(part 1 of 2)
# Autodesk Inventor assembly: gasienica_zlozenie
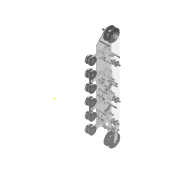
[picture p0: Inventor's stored thumbnail of the model, 180x180]
Saved by Autodesk Inventor 2020.3 (Build 243373000, 373)
## iProperties
Created: 2021-10-24
Part Number: gasienica_zlozenie
Document SubType Name: Assembly
Designer: Patryk Szydlik
Project: Projekt gąsienicowego układu jezdnego robota mobilnego "Ariadna"
Description: Projekt gąsienicowego układu jezdnego robota mobilnego "Ariadna"
Author: Patryk Szydlik
Title: Projekt gąsienicowego układu jezdnego robota mobilnego "Ariadna"
Subject: Projekt gąsienicowego układu jezdnego robota mobilnego "Ariadna"
## Documents named in this file (48)
- C:\Users\patry\Desktop\Semestr 7\Inzynierka\Projekt inventor\Ariadna_inzynierka\Workspaces\Obszar roboczy\Obszar roboczy\Naped\Zawieszenie_v3\gasienica_zlozenie.iam
- C:\Users\patry\Desktop\Semestr 7\Inzynierka\Projekt inventor\Ariadna_inzynierka\Workspaces\Obszar roboczy\Obszar roboczy\Naped\Kola\kolo_przednie.iam
- C:\Users\patry\Desktop\Semestr 7\Inzynierka\Projekt inventor\Ariadna_inzynierka\Workspaces\Obszar roboczy\Obszar roboczy\Naped\Sruby\M5x65.ipt
- C:\Users\patry\Desktop\Semestr 7\Inzynierka\Projekt inventor\Ariadna_inzynierka\Workspaces\Obszar roboczy\Obszar roboczy\Naped\Sruby\M5_nut_5mm.ipt
- C:\Users\patry\Desktop\Semestr 7\Inzynierka\Projekt inventor\Ariadna_inzynierka\Workspaces\Obszar roboczy\Obszar roboczy\Naped\Sruby\dystans_miedzy_plytami.ipt
- C:\Users\patry\Desktop\Semestr 7\Inzynierka\Projekt inventor\Ariadna_inzynierka\Workspaces\Obszar roboczy\Obszar roboczy\Naped\Zawieszenie_v3\tuleja_TUF106040.ipt
- C:\Users\patry\Desktop\Semestr 7\Inzynierka\Projekt inventor\Ariadna_inzynierka\Workspaces\Obszar roboczy\Obszar roboczy\Naped\Sruby\M6_nut_5mm.ipt
- C:\Users\patry\Desktop\Semestr 7\Inzynierka\Projekt inventor\Ariadna_inzynierka\Workspaces\Obszar roboczy\Obszar roboczy\Naped\Amortyzator\Korpus.ipt
- C:\Users\patry\Desktop\Semestr 7\Inzynierka\Projekt inventor\Ariadna_inzynierka\Workspaces\Obszar roboczy\Obszar roboczy\Naped\Amortyzator\Tlok.ipt
- C:\Users\patry\Desktop\Semestr 7\Inzynierka\Projekt inventor\Ariadna_inzynierka\Workspaces\Obszar roboczy\Obszar roboczy\Naped\Amortyzator\Nakretka.ipt
- C:\Users\patry\Desktop\Semestr 7\Inzynierka\Projekt inventor\Ariadna_inzynierka\Workspaces\Obszar roboczy\Obszar roboczy\Naped\Sruby\M8_nut_6.5mm_MIR1.ipt
- C:\Users\patry\Desktop\Semestr 7\Inzynierka\Projekt inventor\Ariadna_inzynierka\Workspaces\Obszar roboczy\Obszar roboczy\Naped\Sruby\M8x80_threaded_MIR1.ipt
- C:\Users\patry\Desktop\Semestr 7\Inzynierka\Projekt inventor\Ariadna_inzynierka\Workspaces\Obszar roboczy\Obszar roboczy\Naped\Sruby\M8_pad_MIR1.ipt
- C:\Users\patry\Desktop\Semestr 7\Inzynierka\Projekt inventor\Ariadna_inzynierka\Workspaces\Obszar roboczy\Obszar roboczy\Naped\Lozyska\608ZZ-8mm\bearings-608zz-80018-1.snapshot.1\608zz_MIR1.ipt
- C:\Users\patry\Desktop\Semestr 7\Inzynierka\Projekt inventor\Ariadna_inzynierka\Workspaces\Obszar roboczy\Obszar roboczy\Naped\Kola\kolo_napedowe.iam
- C:\Users\patry\Desktop\Semestr 7\Inzynierka\Projekt inventor\Ariadna_inzynierka\Workspaces\Obszar roboczy\Obszar roboczy\Naped\Sruby\M5_70_shaft.ipt
- C:\Users\patry\Desktop\Semestr 7\Inzynierka\Projekt inventor\Ariadna_inzynierka\Workspaces\Obszar roboczy\Obszar roboczy\Naped\Sruby\M3_16_shaft.ipt
- C:\Users\patry\Desktop\Semestr 7\Inzynierka\Projekt inventor\Ariadna_inzynierka\Workspaces\Obszar roboczy\Obszar roboczy\Naped\Sruby\M3_nut_2,5mm.ipt
- C:\Users\patry\Desktop\Semestr 7\Inzynierka\Projekt inventor\Ariadna_inzynierka\Workspaces\Obszar roboczy\Obszar roboczy\Naped\Zawieszenie_v3\wspornik_amortyzatora.ipt
- C:\Users\patry\Desktop\Semestr 7\Inzynierka\Projekt inventor\Ariadna_inzynierka\Workspaces\Obszar roboczy\Obszar roboczy\Naped\Sruby\M6_70_shaft.ipt
- C:\Users\patry\Desktop\Semestr 7\Inzynierka\Projekt inventor\Ariadna_inzynierka\Workspaces\Obszar roboczy\Obszar roboczy\Naped\Sruby\tuleja_M5_M9_20.ipt
- C:\Users\patry\Desktop\Semestr 7\Inzynierka\Projekt inventor\Ariadna_inzynierka\Workspaces\Obszar roboczy\Obszar roboczy\Naped\Sruby\tuleja_M5_M9_25.ipt
- C:\Users\patry\Desktop\Semestr 7\Inzynierka\Projekt inventor\Ariadna_inzynierka\Workspaces\Obszar roboczy\Obszar roboczy\Naped\Kola\holder_wheel_pair.iam
- C:\Users\patry\Desktop\Semestr 7\Inzynierka\Projekt inventor\Ariadna_inzynierka\Workspaces\Obszar roboczy\Obszar roboczy\Naped\Zawieszenie_v3\ramie_napinacza.ipt
- C:\Users\patry\Desktop\Semestr 7\Inzynierka\Projekt inventor\Ariadna_inzynierka\Workspaces\Obszar roboczy\Obszar roboczy\Naped\Sruby\M5_60_shaft.ipt
- C:\Users\patry\Desktop\Semestr 7\Inzynierka\Projekt inventor\Ariadna_inzynierka\Workspaces\Obszar roboczy\Obszar roboczy\Naped\Sruby\tuleja_M5_M9_13.ipt
- C:\Users\patry\Desktop\Semestr 7\Inzynierka\Projekt inventor\Ariadna_inzynierka\Workspaces\Obszar roboczy\Obszar roboczy\Naped\Sruby\tuleja_M5_M9_18.ipt
- C:\Users\patry\Desktop\Semestr 7\Inzynierka\Projekt inventor\Ariadna_inzynierka\Workspaces\Obszar roboczy\Obszar roboczy\Naped\Sruby\tuleja_M6_M10_8.ipt
- C:\Users\patry\Desktop\Semestr 7\Inzynierka\Projekt inventor\Ariadna_inzynierka\Workspaces\Obszar roboczy\Obszar roboczy\Naped\Zawieszenie_v3\plyta_boczna.ipt
- C:\Users\patry\Desktop\Semestr 7\Inzynierka\Projekt inventor\Ariadna_inzynierka\Workspaces\Obszar roboczy\Obszar roboczy\Naped\Zawieszenie_v3\ramie_1_wahacza.ipt
- C:\Users\patry\Desktop\Semestr 7\Inzynierka\Projekt inventor\Ariadna_inzynierka\Workspaces\Obszar roboczy\Obszar roboczy\Naped\Zawieszenie_v3\ramie_2_wahacza.ipt
- C:\Users\patry\Desktop\Semestr 7\Inzynierka\Projekt inventor\Ariadna_inzynierka\Workspaces\Obszar roboczy\Obszar roboczy\Naped\Sruby\M6_40_shaft.ipt
- C:\Users\patry\Desktop\Semestr 7\Inzynierka\Projekt inventor\Ariadna_inzynierka\Workspaces\Obszar roboczy\Obszar roboczy\Naped\Sruby\tuleja_M6_M10_7.ipt
- C:\Users\patry\Desktop\Semestr 7\Inzynierka\Projekt inventor\Ariadna_inzynierka\Workspaces\Obszar roboczy\Obszar roboczy\Naped\Sruby\M6_1,25_pad.ipt
- C:\Users\patry\Desktop\Semestr 7\Inzynierka\Projekt inventor\Ariadna_inzynierka\Workspaces\Obszar roboczy\Obszar roboczy\Naped\Sruby\M5_40_shaft.ipt
- M5_shaft.ipt
- C:\Users\patry\Desktop\Semestr 7\Inzynierka\Projekt inventor\Ariadna_inzynierka\Workspaces\Obszar roboczy\Obszar roboczy\Naped\Sruby\tuleja_M5_M9_4,5.ipt
- C:\Users\patry\Desktop\Semestr 7\Inzynierka\Projekt inventor\Ariadna_inzynierka\Workspaces\Obszar roboczy\Obszar roboczy\Naped\Zawieszenie_v3\glowny_wahacz_zewn.ipt
- C:\Users\patry\Desktop\Semestr 7\Inzynierka\Projekt inventor\Ariadna_inzynierka\Workspaces\Obszar roboczy\Obszar roboczy\Naped\Zawieszenie_v3\independent_wheel_pair.iam
- C:\Users\patry\Desktop\Semestr 7\Inzynierka\Projekt inventor\Ariadna_inzynierka\Workspaces\Obszar roboczy\Obszar roboczy\Naped\Sruby\tuleja_M6_M10_6.ipt
- C:\Users\patry\Desktop\Semestr 7\Inzynierka\Projekt inventor\Ariadna_inzynierka\Workspaces\Obszar roboczy\Obszar roboczy\Naped\Sruby\tuleja_M5_M9_17.5.ipt
- C:\Users\patry\Desktop\Semestr 7\Inzynierka\Projekt inventor\Ariadna_inzynierka\Workspaces\Obszar roboczy\Obszar roboczy\Naped\Zawieszenie_v3\komplet_kol_V4.iam
- C:\Users\patry\Desktop\Semestr 7\Inzynierka\Projekt inventor\Ariadna_inzynierka\Workspaces\Obszar roboczy\Obszar roboczy\Naped\Sruby\M6_25_shaft.ipt
- C:\Users\patry\Desktop\Semestr 7\Inzynierka\Projekt inventor\Ariadna_inzynierka\Workspaces\Obszar roboczy\Obszar roboczy\Naped\Kola\single_wheel_dummie.iam
- C:\Users\patry\Desktop\Semestr 7\Inzynierka\Projekt inventor\Ariadna_inzynierka\Workspaces\Obszar roboczy\Obszar roboczy\Naped\Sruby\tuleja_M5_M10_15.ipt
- C:\Users\patry\Desktop\Semestr 7\Inzynierka\Projekt inventor\Ariadna_inzynierka\Workspaces\Obszar roboczy\Obszar roboczy\Naped\Sruby\tuleja_M6_M10_7,5.ipt
- C:\Users\patry\Desktop\Semestr 7\Inzynierka\Projekt inventor\Ariadna_inzynierka\Workspaces\Obszar roboczy\Obszar roboczy\Naped\Zawieszenie_v3\ramie_2_wahacza_tylnego.ipt
- C:\Users\patry\Desktop\Semestr 7\Inzynierka\Projekt inventor\Ariadna_inzynierka\Workspaces\Obszar roboczy\Obszar roboczy\Naped\Sruby\M6x25_plaski_leb.ipt
## Components (346 placed, 46 different names)
1. M5x65:3 — Zestawiające:1808, Zestawiające:1809, Zestawiające:1810
2. M5_nut_5mm:3 — Zestawiające:1810, Zestawiające:1811
3. dystans_miedzy_plytami:3
4. M8_nut_6.5mm_MIR1:1
5. M8x80_threaded_MIR1:1
6. M8_nut_6.5mm_MIR1:2
7. M8_nut_6.5mm_MIR1:3
8. M8_pad_MIR1:1
9. M8_pad_MIR1:2
10. M8_pad_MIR1:3
11. M8_pad_MIR1:4
12. 608zz_MIR1:1
13. 608zz_MIR1:2 — Zestawiające:1077, Równoległe:74
14. kolo_napedowe:1 [sub-assembly]
15. kolo_przednie:1 [sub-assembly]
16. ramie_napinacza:1 — Zestawiające:1807
17. Korpus:6 — Walcowe:6
18. Tlok:6 — Walcowe:6
19. Nakretka:6
20. M5_nut_5mm:34
21. M5_70_shaft:6 — Zestawiające:1080
22. M5_nut_5mm:35
23. M3_16_shaft:6
24. M3_nut_2,5mm:11
25. M3_nut_2,5mm:12
26. wspornik_amortyzatora:11 — Zestawiające:1086, Zestawiające:1087
27. wspornik_amortyzatora:12
28. M5_nut_5mm:36
29. M5_nut_5mm:37
30. M5_nut_5mm:38
31. M5_nut_5mm:39
32. tuleja_M5_M9_20:6
33. tuleja_M5_M9_25:6
34. ramie_napinacza:2 — Zestawiające:1804
35. M5_60_shaft:1 — Zestawiające:1086
36. M5_60_shaft:2 — Zestawiające:1087, Zestawiające:1796, Zestawiające:1797
37. tuleja_TUF106040:41 — Zestawiające:1085
38. tuleja_TUF106040:42
39. M6_70_shaft:11 — Zestawiające:1079, Zestawiające:1802, Zestawiające:1803, Zestawiające:1806
40. M6_nut_5mm:49
41. M6_nut_5mm:50
42. tuleja_M5_M9_13:1 — Zestawiające:1796
43. tuleja_M5_M9_18:1 — Zestawiające:1797
44. M6_70_shaft:12
45. M6_nut_5mm:51
46. M6_nut_5mm:52
47. tuleja_M6_M10_8:1
48. tuleja_M6_M10_8:2
49. holder_wheel_pair:4 [sub-assembly] — Zestawiające:1082, Zestawiające:1083
50. holder_wheel_pair:5 [sub-assembly] — Zestawiające:1081, Zestawiające:1084
51. plyta_boczna:1 — Zestawiające:1075, Zestawiające:1076, Zestawiające:1077, Zestawiające:1078, Równoległe:74, Kątowe:22, Zestawiające:1079, Zestawiające:1080, Zestawiające:1081, Zestawiające:1082, Zestawiające:1083, Zestawiające:1084, Zestawiające:1085, Zestawiające:1632, Zestawiające:1633, Kątowe:49, Zestawiające:1808, Zestawiające:1809, Zestawiające:1950, Zestawiające:1951, Zestawiające:1952, Zestawiające:1953
52. plyta_boczna:2 — Zestawiające:1075, Zestawiające:1076, Zestawiające:1078, Zestawiające:1636, Zestawiające:1637, Zestawiające:1638, Zestawiające:1639, Zestawiające:1640, Zestawiające:1641, Zestawiające:1777, Zestawiające:1778, Zestawiające:1779, Zestawiające:1780, Zestawiające:1811
53. ramie_1_wahacza:3
54. ramie_2_wahacza:3
55. tuleja_TUF106040:51
56. tuleja_TUF106040:52
57. tuleja_TUF106040:53
58. tuleja_TUF106040:54
59. tuleja_TUF106040:55
60. tuleja_TUF106040:56
61. ramie_2_wahacza:4
62. tuleja_TUF106040:57
63. tuleja_TUF106040:58
64. M6_nut_5mm:65
65. Korpus:8
66. Tlok:8
67. Nakretka:8
68. M5_nut_5mm:48
69. M5_70_shaft:8
70. ramie_1_wahacza:4 — Kątowe:40
71. M5_nut_5mm:49
72. M3_16_shaft:8
73. M3_nut_2,5mm:15
74. M3_nut_2,5mm:16
75. wspornik_amortyzatora:15
76. wspornik_amortyzatora:16
77. M6_40_shaft:3
78. M6_40_shaft:4
79. M6_nut_5mm:66
80. M6_nut_5mm:67
81. M6_nut_5mm:68
82. tuleja_M6_M10_7:4
83. tuleja_M6_M10_7:5
84. M6_1,25_pad:9
85. M6_1,25_pad:10
86. M6_1,25_pad:11
87. M6_1,25_pad:12
88. M6_1,25_pad:13
89. M6_1,25_pad:14
90. M6_1,25_pad:15
91. M6_1,25_pad:16
92. M6_70_shaft:15 — Zestawiające:1636
93. M6_70_shaft:16 — Zestawiające:1632
94. M6_nut_5mm:69
95. M6_nut_5mm:70
96. M6_nut_5mm:71
97. M6_nut_5mm:72
98. M5_shaft:3
99. M5_shaft:4
100. M5_nut_5mm:50
101. M5_nut_5mm:51
102. M5_nut_5mm:52
103. M5_nut_5mm:53
104. tuleja_M5_M9_4,5:5
105. tuleja_M5_M9_4,5:6
106. tuleja_M5_M9_4,5:7
107. tuleja_M5_M9_4,5:8
108. lacznik_zewn:3 — Kątowe:40, Zestawiające:1793, Zestawiające:1794, Zestawiające:1795
109. lacznik_zewn:4 — Zestawiające:1793
110. tuleja_M6_M10_6:5
111. M6_nut_5mm:73
112. M6_nut_5mm:74
113. M6_nut_5mm:75 — Zestawiające:1633
114. M6_nut_5mm:76
115. tuleja_M6_M10_6:6
116. tuleja_M6_M10_6:7
117. tuleja_M6_M10_6:8
118. M5_nut_5mm:54
119. M5_nut_5mm:55
120. tuleja_M5_M9_17.5:3 — Zestawiające:1637
121. tuleja_M5_M9_17.5:4
122. ramie_1_wahacza:7 — Kątowe:41
123. ramie_2_wahacza:7
124. tuleja_TUF106040:67
125. tuleja_TUF106040:68
126. tuleja_TUF106040:69
127. tuleja_TUF106040:70
128. tuleja_TUF106040:71
129. tuleja_TUF106040:72
130. ramie_2_wahacza:8
131. tuleja_TUF106040:73
132. tuleja_TUF106040:74
133. M6_nut_5mm:89
134. Korpus:10 — Walcowe:10
135. Tlok:10 — Walcowe:10
136. Nakretka:10
137. M5_nut_5mm:64
138. M5_70_shaft:10
139. ramie_1_wahacza:8
140. M5_nut_5mm:65 — Zestawiające:1638
141. M3_16_shaft:10
142. M3_nut_2,5mm:19
143. M3_nut_2,5mm:20
144. wspornik_amortyzatora:19
145. wspornik_amortyzatora:20
146. M6_40_shaft:7
147. M6_40_shaft:8
148. M6_nut_5mm:90
149. M6_nut_5mm:91
150. M6_nut_5mm:92
151. tuleja_M6_M10_7:10
152. tuleja_M6_M10_7:11
153. M6_1,25_pad:25
154. M6_1,25_pad:26
155. M6_1,25_pad:27
156. M6_1,25_pad:28
157. M6_1,25_pad:29
158. M6_1,25_pad:30
159. M6_1,25_pad:31
160. M6_1,25_pad:32
161. M6_70_shaft:19 — Zestawiające:1640
162. M6_70_shaft:20 — Zestawiające:1639
163. M6_nut_5mm:93
164. M6_nut_5mm:94
165. M6_nut_5mm:95
166. M6_nut_5mm:96
167. M5_shaft:7
168. M5_shaft:8
169. M5_nut_5mm:66
170. M5_nut_5mm:67
171. M5_nut_5mm:68
172. M5_nut_5mm:69
173. tuleja_M5_M9_4,5:13
174. tuleja_M5_M9_4,5:14
175. tuleja_M5_M9_4,5:15
176. tuleja_M5_M9_4,5:16
177. lacznik_zewn:7 — Zestawiające:1784
178. lacznik_zewn:8 — Kątowe:41, Zestawiające:1781, Zestawiające:1782, Zestawiające:1789
179. tuleja_M6_M10_6:13
180. M6_nut_5mm:97
181. M6_nut_5mm:98
182. M6_nut_5mm:99
183. M6_nut_5mm:100
184. tuleja_M6_M10_6:14
185. tuleja_M6_M10_6:15
186. tuleja_M6_M10_6:16
187. M5_nut_5mm:70
188. M5_nut_5mm:71
189. tuleja_M5_M9_17.5:7 — Zestawiające:1641
190. tuleja_M5_M9_17.5:8
191. ramie_1_wahacza:9 — Kątowe:47
192. ramie_2_wahacza:9
193. tuleja_TUF106040:75
194. tuleja_TUF106040:76
195. tuleja_TUF106040:77
196. tuleja_TUF106040:78
197. tuleja_TUF106040:79
198. tuleja_TUF106040:80
199. ramie_2_wahacza:10
200. tuleja_TUF106040:81
201. tuleja_TUF106040:82
202. M6_nut_5mm:101
203. Korpus:11 — Walcowe:11
204. Tlok:11 — Walcowe:11
205. Nakretka:11
206. M5_nut_5mm:72
207. M5_70_shaft:11
208. ramie_1_wahacza:10
209. M5_nut_5mm:73
210. M3_16_shaft:11
211. M3_nut_2,5mm:21
212. M3_nut_2,5mm:22
213. wspornik_amortyzatora:21
214. wspornik_amortyzatora:22
215. M6_40_shaft:9
216. M6_40_shaft:10
217. M6_nut_5mm:102
218. M6_nut_5mm:103
219. M6_nut_5mm:104
220. tuleja_M6_M10_7:13
221. tuleja_M6_M10_7:14
222. M6_1,25_pad:33
223. M6_1,25_pad:34
224. M6_1,25_pad:35
225. M6_1,25_pad:36
226. M6_1,25_pad:37
227. M6_1,25_pad:38
228. M6_1,25_pad:39
229. M6_1,25_pad:40
230. M6_70_shaft:21 — Zestawiające:1779
231. M6_70_shaft:22 — Zestawiające:1778
232. M6_nut_5mm:105
233. M6_nut_5mm:106
234. M6_nut_5mm:107 — Zestawiające:1777
235. M6_nut_5mm:108
236. M5_shaft:9
237. M5_shaft:10
238. M5_nut_5mm:74
239. M5_nut_5mm:75
240. M5_nut_5mm:76
241. M5_nut_5mm:77
242. tuleja_M5_M9_4,5:17
243. tuleja_M5_M9_4,5:18
244. tuleja_M5_M9_4,5:19
245. tuleja_M5_M9_4,5:20
246. lacznik_zewn:9
247. lacznik_zewn:10 — Kątowe:47
248. independent_wheel_pair:5 [sub-assembly]
249. tuleja_M6_M10_7:15
250. tuleja_M6_M10_6:17
251. M6_nut_5mm:109
252. M6_nut_5mm:110
253. M6_nut_5mm:111
254. M6_nut_5mm:112
255. tuleja_M6_M10_6:18
256. tuleja_M6_M10_6:19
257. tuleja_M6_M10_6:20
258. M5_nut_5mm:78
259. M5_nut_5mm:79
260. tuleja_M5_M9_17.5:9
261. tuleja_M5_M9_17.5:10 — Zestawiające:1780
262. komplet_kol_V4:1 [sub-assembly] — Zestawiające:1781, Zestawiające:1782, Zestawiające:1784, Zestawiające:1788, Kątowe:48
263. M6_nut_5mm:115 — Zestawiające:1789
264. M6_25_shaft:2 — Zestawiające:1788
265. M6_nut_5mm:116
266. komplet_kol_V4:2 [sub-assembly] — Zestawiające:1795, Kątowe:48, Kątowe:49, Styczny:1
267. M6_nut_5mm:117
268. M6_25_shaft:3 — Zestawiające:1794
269. M6_nut_5mm:118
270. single_wheel_dummie:1 [sub-assembly] — Zestawiające:1799
271. single_wheel_dummie:2 [sub-assembly] — Zestawiające:1800, Zestawiające:1801, Zestawiające:1802, Zestawiające:1805
272. tuleja_M5_M10_15:1 — Zestawiające:1799, Zestawiające:1800, Zestawiające:1801
273. tuleja_M6_M10_7,5:1 — Zestawiające:1803, Zestawiające:1804, Zestawiające:1805
274. tuleja_M6_M10_7,5:2 — Zestawiające:1806, Zestawiające:1807
275. ramie_1_wahacza:11
276. tuleja_TUF106040:83
277. tuleja_TUF106040:84
278. tuleja_TUF106040:85
279. tuleja_TUF106040:86
280. tuleja_TUF106040:87
281. tuleja_TUF106040:88
282. tuleja_TUF106040:89
283. tuleja_TUF106040:90
284. M6_nut_5mm:119
285. Korpus:12 — Walcowe:12
286. Tlok:12 — Walcowe:12
287. Nakretka:12
288. M5_nut_5mm:80
289. M5_70_shaft:12
290. ramie_1_wahacza:12
291. M5_nut_5mm:81
292. M3_16_shaft:12
293. M3_nut_2,5mm:23
294. M3_nut_2,5mm:24
295. wspornik_amortyzatora:23
296. wspornik_amortyzatora:24
297. M6_40_shaft:11
298. M6_40_shaft:12
299. M6_nut_5mm:120
300. M6_nut_5mm:121
301. M6_nut_5mm:122
302. tuleja_M6_M10_7:16
303. tuleja_M6_M10_7:17
304. M6_1,25_pad:41
305. M6_1,25_pad:42
306. M6_1,25_pad:43
307. M6_1,25_pad:44
308. M6_1,25_pad:45
309. M6_1,25_pad:46
310. M6_1,25_pad:47
311. M6_1,25_pad:48
312. M6_70_shaft:23 — Zestawiające:1950
313. M6_nut_5mm:123 — Zestawiające:1951
314. M6_nut_5mm:124
315. M6_nut_5mm:125
316. M6_nut_5mm:126
317. M5_shaft:11
318. M5_shaft:12
319. M5_nut_5mm:82
320. M5_nut_5mm:83
321. M5_nut_5mm:84
322. M5_nut_5mm:85
323. tuleja_M5_M9_4,5:21
324. tuleja_M5_M9_4,5:22
325. tuleja_M5_M9_4,5:23
326. tuleja_M5_M9_4,5:24
327. lacznik_zewn:11
328. lacznik_zewn:12
329. independent_wheel_pair:6 [sub-assembly] — Styczny:1
330. tuleja_M6_M10_7:18
331. tuleja_M6_M10_6:21
332. M6_nut_5mm:127
333. M6_nut_5mm:128
334. M6_nut_5mm:129
335. M6_nut_5mm:130
336. tuleja_M6_M10_6:22 — Zestawiające:1952
337. tuleja_M6_M10_6:23
338. tuleja_M6_M10_6:24
339. M5_nut_5mm:86
340. M5_nut_5mm:87
341. tuleja_M5_M9_17.5:11
342. tuleja_M5_M9_17.5:12 — Zestawiające:1953
343. ramie_2_wahacza_tylnego:1
344. ramie_2_wahacza_tylnego:2
345. M6x25_plaski_leb:1
346. M6x25_plaski_leb:2
## Relationships (744: Mate 670, Flush 48, Angle 21, CylindricalJoint 4, Tangent 1)
- [Mate]: M5x65:3 ↔ dystans_miedzy_plytami:3
- [Mate] (5 mm): M5x65:3 ↔ dystans_miedzy_plytami:3
- [Mate]: M8_nut_6.5mm_MIR1:1 ↔ M8x80_threaded_MIR1:1
- [Mate]: M8x80_threaded_MIR1:1 ↔ M8_nut_6.5mm_MIR1:2
- [Mate]: M8x80_threaded_MIR1:1 ↔ M8_nut_6.5mm_MIR1:3
- [Mate]: M8_nut_6.5mm_MIR1:1 ↔ M8_pad_MIR1:1
- [Mate] (7 mm): M8x80_threaded_MIR1:1 ↔ M8_pad_MIR1:1
- [Mate]: M8x80_threaded_MIR1:1 ↔ M8_pad_MIR1:1
- [Mate]: M8_nut_6.5mm_MIR1:1 ↔ M8_pad_MIR1:2
- [Mate]: M8x80_threaded_MIR1:1 ↔ M8_pad_MIR1:2
- [Mate] (7 mm): M8_nut_6.5mm_MIR1:2 ↔ M8_pad_MIR1:3
- [Mate]: M8_nut_6.5mm_MIR1:3 ↔ M8_pad_MIR1:3
- [Mate]: M8x80_threaded_MIR1:1 ↔ M8_pad_MIR1:3
- [Mate]: M8_nut_6.5mm_MIR1:3 ↔ M8_pad_MIR1:4
- [Mate] (31 mm): M8_pad_MIR1:2 ↔ M8_pad_MIR1:4
- [Mate]: M8x80_threaded_MIR1:1 ↔ M8_pad_MIR1:4
- [Mate]: M8x80_threaded_MIR1:1 ↔ 608zz_MIR1:1
- [Mate]: M8_nut_6.5mm_MIR1:2 ↔ 608zz_MIR1:1
- [Mate]: M8x80_threaded_MIR1:1 ↔ 608zz_MIR1:2
- [Mate]: M8x80_threaded_MIR1:1 ↔ 608zz_MIR1:2
- [Mate]: M8x80_threaded_MIR1:1 ↔ kolo_napedowe:1
- [Mate]: M8_pad_MIR1:2 ↔ kolo_napedowe:1
- [Mate]: Korpus:6 ↔ Tlok:6
- [Angle] (0 deg): Korpus:6 ↔ Tlok:6
- [Mate]: Korpus:6 ↔ Nakretka:6
- [Mate] (5 mm): Korpus:6 ↔ Nakretka:6
- Walcowe:6 [CylindricalJoint]: Korpus:6 ↔ Tlok:6
- [Mate]: Korpus:6 ↔ M5_70_shaft:6
- [Flush] (-30 mm): Korpus:6 ↔ M5_70_shaft:6
- [Mate]: M5_nut_5mm:34 ↔ M5_70_shaft:6
- [Mate]: M5_70_shaft:6 ↔ M5_nut_5mm:35
- [Mate] (60 mm): M5_nut_5mm:34 ↔ M5_nut_5mm:35
- [Mate] (30 mm): Korpus:6 ↔ M5_nut_5mm:34
- [Mate]: wspornik_amortyzatora:11 ↔ wspornik_amortyzatora:12
- [Mate]: wspornik_amortyzatora:11 ↔ wspornik_amortyzatora:12
- [Mate] (5 mm): wspornik_amortyzatora:11 ↔ wspornik_amortyzatora:12
- [Mate]: M3_16_shaft:6 ↔ wspornik_amortyzatora:12
- [Flush] (-2.5 mm): M3_16_shaft:6 ↔ wspornik_amortyzatora:11
- [Mate]: M3_16_shaft:6 ↔ M3_nut_2,5mm:11
- [Mate]: M3_nut_2,5mm:11 ↔ wspornik_amortyzatora:11
- [Mate]: M3_16_shaft:6 ↔ M3_nut_2,5mm:12
- [Mate]: M3_nut_2,5mm:12 ↔ wspornik_amortyzatora:12
- [Mate]: Tlok:6 ↔ M3_16_shaft:6
- [Mate]: Tlok:6 ↔ wspornik_amortyzatora:12
- [Mate]: M5_70_shaft:6 ↔ tuleja_M5_M9_20:6
- [Mate]: Korpus:6 ↔ tuleja_M5_M9_20:6
- [Mate]: M5_70_shaft:6 ↔ tuleja_M5_M9_25:6
- [Mate]: Korpus:6 ↔ tuleja_M5_M9_25:6
- [Mate]: M6_70_shaft:11 ↔ M6_nut_5mm:49
- [Mate]: M6_70_shaft:11 ↔ M6_nut_5mm:50
- [Mate] (60 mm): M6_nut_5mm:49 ↔ M6_nut_5mm:50
- [Mate]: tuleja_TUF106040:41 ↔ M6_70_shaft:11
- [Mate]: ramie_napinacza:1 ↔ ramie_napinacza:2
- [Mate]: ramie_napinacza:1 ↔ ramie_napinacza:2
- [Mate] (42 mm): ramie_napinacza:1 ↔ ramie_napinacza:2
- [Mate]: ramie_napinacza:1 ↔ tuleja_TUF106040:41
- [Mate]: ramie_napinacza:1 ↔ tuleja_TUF106040:41
- [Mate]: ramie_napinacza:2 ↔ tuleja_TUF106040:42
- [Mate]: ramie_napinacza:2 ↔ tuleja_TUF106040:42
- [Mate] (5 mm): tuleja_TUF106040:41 ↔ M6_nut_5mm:49
- [Flush] (-11 mm): ramie_napinacza:2 ↔ M6_70_shaft:11
- [Mate] (5.5 mm): kolo_przednie:1 ↔ ramie_napinacza:1
- [Mate]: kolo_przednie:1 ↔ ramie_napinacza:1
- [Mate]: ramie_napinacza:1 ↔ M5_60_shaft:1
- [Flush] (6 mm): ramie_napinacza:1 ↔ M5_60_shaft:1
- [Mate]: ramie_napinacza:1 ↔ M5_60_shaft:2
- [Flush] (6 mm): ramie_napinacza:1 ↔ M5_60_shaft:2
- [Mate]: M5_nut_5mm:37 ↔ M5_60_shaft:1
- [Mate]: ramie_napinacza:1 ↔ M5_nut_5mm:37
- [Mate]: M5_nut_5mm:38 ↔ M5_60_shaft:1
- [Mate]: M5_nut_5mm:38 ↔ ramie_napinacza:2
- [Mate]: M5_nut_5mm:39 ↔ M5_60_shaft:2
- [Mate]: M5_nut_5mm:39 ↔ ramie_napinacza:2
- [Mate]: M5_nut_5mm:36 ↔ M5_60_shaft:2
- [Mate]: ramie_napinacza:1 ↔ M5_nut_5mm:36
- [Flush]: M5_nut_5mm:34 ↔ M6_nut_5mm:50
- [Mate]: wspornik_amortyzatora:12 ↔ tuleja_M5_M9_18:1
- [Mate]: ramie_napinacza:1 ↔ tuleja_M5_M9_13:1
- [Mate]: ramie_napinacza:1 ↔ M6_70_shaft:12
- [Flush] (-11 mm): ramie_napinacza:1 ↔ M6_70_shaft:12
- [Mate]: M6_70_shaft:12 ↔ M6_nut_5mm:51
- [Mate]: ramie_napinacza:1 ↔ M6_nut_5mm:51
- [Mate]: M6_70_shaft:12 ↔ M6_nut_5mm:52
- [Mate]: ramie_napinacza:2 ↔ M6_nut_5mm:52
- [Mate]: M6_70_shaft:12 ↔ tuleja_M6_M10_8:1
- [Mate]: ramie_napinacza:1 ↔ tuleja_M6_M10_8:1
- [Mate]: M6_70_shaft:12 ↔ tuleja_M6_M10_8:2
- [Mate]: ramie_napinacza:2 ↔ tuleja_M6_M10_8:2
- Zestawiające:1075 [Mate]: plyta_boczna:1 ↔ plyta_boczna:2
- Zestawiające:1076 [Mate]: plyta_boczna:1 ↔ plyta_boczna:2
- Zestawiające:1077 [Mate]: 608zz_MIR1:2 ↔ plyta_boczna:1
- Zestawiające:1078 [Mate] (50 mm): plyta_boczna:1 ↔ plyta_boczna:2
- Równoległe:74 [Flush] (-1 mm): 608zz_MIR1:2 ↔ plyta_boczna:1
- Kątowe:22 [Angle] (180 deg): plyta_boczna:1
- Zestawiające:1079 [Mate]: M6_70_shaft:11 ↔ plyta_boczna:1
- Zestawiające:1080 [Mate]: M5_70_shaft:6 ↔ plyta_boczna:1
- Zestawiające:1081 [Mate]: holder_wheel_pair:5 ↔ plyta_boczna:1
- Zestawiające:1082 [Mate]: holder_wheel_pair:4 ↔ plyta_boczna:1
- Zestawiające:1083 [Mate]: holder_wheel_pair:4 ↔ plyta_boczna:1
- Zestawiające:1084 [Mate]: holder_wheel_pair:5 ↔ plyta_boczna:1
- Zestawiające:1085 [Mate]: tuleja_TUF106040:41 ↔ plyta_boczna:1
- Zestawiające:1086 [Mate]: wspornik_amortyzatora:11 ↔ M5_60_shaft:1
- Zestawiające:1087 [Mate]: wspornik_amortyzatora:11 ↔ M5_60_shaft:2
- [Mate]: ramie_2_wahacza:3 ↔ tuleja_TUF106040:51
- [Mate]: ramie_2_wahacza:3 ↔ tuleja_TUF106040:51
- [Angle] (0 deg): ramie_2_wahacza:3 ↔ tuleja_TUF106040:51
- [Mate]: ramie_1_wahacza:3 ↔ tuleja_TUF106040:54
- [Mate]: ramie_1_wahacza:3 ↔ tuleja_TUF106040:54
- [Angle] (0 deg): ramie_1_wahacza:3 ↔ tuleja_TUF106040:54
- [Mate]: ramie_2_wahacza:4 ↔ tuleja_TUF106040:57
- [Mate]: ramie_2_wahacza:4 ↔ tuleja_TUF106040:57
- [Angle] (0 deg): ramie_2_wahacza:4 ↔ tuleja_TUF106040:57
- [Mate]: Korpus:8 ↔ Tlok:8
- [Angle] (0 deg): Korpus:8 ↔ Tlok:8
- [Mate]: Korpus:8 ↔ Nakretka:8
- [Mate] (5 mm): Korpus:8 ↔ Nakretka:8
- [Mate]: Korpus:8 ↔ M5_70_shaft:8
- [Flush] (-32.5 mm): Korpus:8 ↔ M5_70_shaft:8
- [Mate]: M5_nut_5mm:48 ↔ M5_70_shaft:8
- [Mate]: M5_70_shaft:8 ↔ M5_nut_5mm:49
- [Mate] (60 mm): M5_nut_5mm:48 ↔ M5_nut_5mm:49
- [Mate] (27.5 mm): Korpus:8 ↔ M5_nut_5mm:48
- [Mate]: tuleja_TUF106040:56 ↔ ramie_1_wahacza:4
- [Mate]: tuleja_TUF106040:55 ↔ ramie_1_wahacza:4
- [Mate]: tuleja_TUF106040:56 ↔ ramie_1_wahacza:4
- [Mate]: tuleja_TUF106040:51 ↔ tuleja_TUF106040:57
- [Mate]: wspornik_amortyzatora:15 ↔ wspornik_amortyzatora:16
- [Mate]: wspornik_amortyzatora:15 ↔ wspornik_amortyzatora:16
- [Mate] (5 mm): wspornik_amortyzatora:15 ↔ wspornik_amortyzatora:16
- [Mate]: M3_16_shaft:8 ↔ wspornik_amortyzatora:16
- [Flush] (-2.5 mm): M3_16_shaft:8 ↔ wspornik_amortyzatora:15
- [Mate]: M3_16_shaft:8 ↔ M3_nut_2,5mm:15
- [Mate]: M3_nut_2,5mm:15 ↔ wspornik_amortyzatora:15
- [Mate]: M3_16_shaft:8 ↔ M3_nut_2,5mm:16
- [Mate]: M3_nut_2,5mm:16 ↔ wspornik_amortyzatora:16
- [Mate]: Tlok:8 ↔ M3_16_shaft:8
- [Mate]: Tlok:8 ↔ wspornik_amortyzatora:16
- [Mate]: ramie_1_wahacza:3 ↔ wspornik_amortyzatora:15
- [Mate]: ramie_1_wahacza:3 ↔ wspornik_amortyzatora:15
- [Mate] (4.5 mm): ramie_1_wahacza:3 ↔ wspornik_amortyzatora:15
- [Mate]: tuleja_TUF106040:54 ↔ M6_40_shaft:3
- [Flush] (7 mm): ramie_1_wahacza:3 ↔ M6_40_shaft:3
- [Mate]: tuleja_TUF106040:57 ↔ M6_40_shaft:4
- [Flush] (7 mm): ramie_2_wahacza:4 ↔ M6_40_shaft:4
- [Mate]: M6_nut_5mm:65 ↔ M6_40_shaft:3
- [Mate]: ramie_1_wahacza:3 ↔ M6_nut_5mm:65
- [Mate]: M6_40_shaft:3 ↔ M6_nut_5mm:66
- [Mate]: ramie_1_wahacza:4 ↔ M6_nut_5mm:66
- [Mate]: M6_40_shaft:4 ↔ M6_nut_5mm:67
- [Mate]: ramie_2_wahacza:3 ↔ M6_nut_5mm:67
- [Mate]: M6_40_shaft:4 ↔ M6_nut_5mm:68
- [Mate]: ramie_2_wahacza:4 ↔ M6_nut_5mm:68
- [Mate]: M6_40_shaft:3 ↔ tuleja_M6_M10_7:4
- [Mate]: M6_40_shaft:4 ↔ tuleja_M6_M10_7:5
- [Mate]: M6_1,25_pad:9 ↔ M6_1,25_pad:10
- [Mate]: M6_1,25_pad:9 ↔ M6_1,25_pad:10
- [Mate]: M6_40_shaft:3 ↔ M6_1,25_pad:9
- [Mate]: M6_1,25_pad:11 ↔ M6_1,25_pad:12
- [Mate]: M6_1,25_pad:11 ↔ M6_1,25_pad:12
- [Mate]: M6_40_shaft:3 ↔ M6_1,25_pad:11
- [Mate]: tuleja_TUF106040:54 ↔ M6_1,25_pad:11
- [Mate]: M6_1,25_pad:13 ↔ M6_1,25_pad:14
- [Mate]: M6_1,25_pad:13 ↔ M6_1,25_pad:14
- [Mate]: M6_40_shaft:4 ↔ M6_1,25_pad:13
- [Mate]: M6_1,25_pad:15 ↔ M6_1,25_pad:16
- [Mate]: M6_1,25_pad:15 ↔ M6_1,25_pad:16
- [Mate]: M6_40_shaft:4 ↔ M6_1,25_pad:15
- [Mate]: tuleja_TUF106040:57 ↔ M6_1,25_pad:15
- [Mate]: M5_70_shaft:8 ↔ M6_70_shaft:15
- [Flush]: M5_70_shaft:8 ↔ M6_70_shaft:16
- [Mate]: M6_70_shaft:16 ↔ M6_nut_5mm:69
- [Mate]: M6_70_shaft:16 ↔ M6_nut_5mm:70
- [Mate] (60 mm): M6_nut_5mm:69 ↔ M6_nut_5mm:70
- [Flush]: M5_nut_5mm:48 ↔ M6_nut_5mm:70
- [Mate] (60 mm): M6_nut_5mm:71 ↔ M6_nut_5mm:72
- [Mate]: M6_nut_5mm:71 ↔ M6_nut_5mm:72
- [Mate]: M6_70_shaft:15 ↔ M6_nut_5mm:71
- [Flush]: M5_nut_5mm:48 ↔ M6_nut_5mm:72
- [Mate]: ramie_1_wahacza:3 ↔ M5_shaft:3
- [Flush] (7 mm): ramie_1_wahacza:3 ↔ M5_shaft:3
- [Mate]: ramie_1_wahacza:3 ↔ M5_shaft:4
- [Flush] (7 mm): ramie_1_wahacza:3 ↔ M5_shaft:4
- [Mate]: M5_shaft:4 ↔ M5_nut_5mm:50
- [Mate]: ramie_1_wahacza:3 ↔ M5_nut_5mm:50
- [Mate]: M5_shaft:3 ↔ M5_nut_5mm:51
- [Mate]: ramie_1_wahacza:3 ↔ M5_nut_5mm:51
- [Mate]: M5_shaft:3 ↔ M5_nut_5mm:52
- [Mate]: ramie_1_wahacza:4 ↔ M5_nut_5mm:52
- [Mate]: M5_shaft:4 ↔ M5_nut_5mm:53
- [Mate]: ramie_1_wahacza:4 ↔ M5_nut_5mm:53
- [Mate]: M5_shaft:3 ↔ tuleja_M5_M9_4,5:5
- [Mate]: ramie_1_wahacza:4 ↔ tuleja_M5_M9_4,5:5
- [Mate]: M5_shaft:3 ↔ tuleja_M5_M9_4,5:6
- [Mate]: ramie_1_wahacza:3 ↔ tuleja_M5_M9_4,5:6
- [Mate]: M5_shaft:4 ↔ tuleja_M5_M9_4,5:7
- [Mate]: ramie_1_wahacza:4 ↔ tuleja_M5_M9_4,5:7
- [Mate]: M5_shaft:4 ↔ tuleja_M5_M9_4,5:8
- [Mate]: ramie_1_wahacza:3 ↔ tuleja_M5_M9_4,5:8
- [Mate]: M6_40_shaft:4 ↔ lacznik_zewn:3
- [Mate]: tuleja_M6_M10_7:5 ↔ lacznik_zewn:3
- [Mate]: M6_40_shaft:3 ↔ lacznik_zewn:3
- [Mate]: M6_40_shaft:4 ↔ lacznik_zewn:4
- [Mate]: M6_40_shaft:3 ↔ lacznik_zewn:4
- [Mate]: tuleja_TUF106040:56 ↔ M6_40_shaft:3
- [Mate]: M6_1,25_pad:12 ↔ lacznik_zewn:4
- [Mate]: M6_1,25_pad:16 ↔ lacznik_zewn:4
- [Mate]: tuleja_M6_M10_7:4 ↔ lacznik_zewn:3
- [Mate]: M6_1,25_pad:9 ↔ lacznik_zewn:3
- [Mate]: tuleja_TUF106040:56 ↔ M6_1,25_pad:10
- [Mate]: M6_1,25_pad:13 ↔ lacznik_zewn:3
- [Mate]: tuleja_TUF106040:51 ↔ M6_1,25_pad:14
- [Mate]: tuleja_TUF106040:55 ↔ ramie_1_wahacza:4
- [Mate]: tuleja_TUF106040:53 ↔ M6_70_shaft:16
- [Mate]: ramie_1_wahacza:3 ↔ tuleja_TUF106040:53
- [Mate]: ramie_1_wahacza:3 ↔ tuleja_TUF106040:53
- [Mate]: tuleja_TUF106040:52 ↔ M6_70_shaft:15
- [Mate]: ramie_2_wahacza:3 ↔ tuleja_TUF106040:52
- [Mate]: ramie_2_wahacza:3 ↔ tuleja_TUF106040:52
- [Mate]: tuleja_TUF106040:58 ↔ M6_70_shaft:15
- [Mate]: ramie_2_wahacza:4 ↔ tuleja_TUF106040:58
- [Mate]: ramie_2_wahacza:4 ↔ tuleja_TUF106040:58
- [Mate]: ramie_1_wahacza:4 ↔ M5_shaft:4
- [Mate]: M6_70_shaft:15 ↔ M6_nut_5mm:73
- [Mate] (5 mm): M6_nut_5mm:72 ↔ M6_nut_5mm:73
- [Mate]: M6_70_shaft:15 ↔ M6_nut_5mm:74
- [Mate] (5 mm): M6_nut_5mm:71 ↔ M6_nut_5mm:74
- [Mate]: M6_70_shaft:16 ↔ M6_nut_5mm:75
- [Mate] (5 mm): M6_nut_5mm:69 ↔ M6_nut_5mm:75
- [Mate]: M6_70_shaft:16 ↔ M6_nut_5mm:76
- [Mate] (5 mm): M6_nut_5mm:70 ↔ M6_nut_5mm:76
- [Mate]: M6_70_shaft:16 ↔ tuleja_M6_M10_6:5
- [Mate]: tuleja_M6_M10_6:5 ↔ M6_nut_5mm:75
- [Mate]: M6_70_shaft:15 ↔ tuleja_M6_M10_6:6
- [Mate]: tuleja_TUF106040:58 ↔ tuleja_M6_M10_6:6
- [Mate]: M6_70_shaft:15 ↔ tuleja_M6_M10_6:7
- [Mate]: tuleja_TUF106040:52 ↔ tuleja_M6_M10_6:7
- [Mate]: M6_70_shaft:16 ↔ tuleja_M6_M10_6:8
- [Mate]: tuleja_TUF106040:55 ↔ tuleja_M6_M10_6:8
- [Mate]: M5_70_shaft:8 ↔ M5_nut_5mm:54
- [Mate] (5 mm): M5_nut_5mm:48 ↔ M5_nut_5mm:54
- [Mate]: M5_70_shaft:8 ↔ M5_nut_5mm:55
- [Mate] (5 mm): M5_nut_5mm:49 ↔ M5_nut_5mm:55
- [Mate]: M5_70_shaft:8 ↔ tuleja_M5_M9_17.5:4
- [Mate]: M5_nut_5mm:55 ↔ tuleja_M5_M9_17.5:4
- [Mate]: M5_70_shaft:8 ↔ tuleja_M5_M9_17.5:3
- [Mate]: Korpus:8 ↔ tuleja_M5_M9_17.5:3
- [Mate]: ramie_2_wahacza:7 ↔ tuleja_TUF106040:67
- [Mate]: ramie_2_wahacza:7 ↔ tuleja_TUF106040:67
- [Angle] (0 deg): ramie_2_wahacza:7 ↔ tuleja_TUF106040:67
- [Mate]: ramie_1_wahacza:7 ↔ tuleja_TUF106040:70
- [Mate]: ramie_1_wahacza:7 ↔ tuleja_TUF106040:70
- [Angle] (0 deg): ramie_1_wahacza:7 ↔ tuleja_TUF106040:70
- [Mate]: ramie_2_wahacza:8 ↔ tuleja_TUF106040:73
- [Mate]: ramie_2_wahacza:8 ↔ tuleja_TUF106040:73
- [Angle] (0 deg): ramie_2_wahacza:8 ↔ tuleja_TUF106040:73
- [Mate]: Korpus:10 ↔ Tlok:10
- [Angle] (0 deg): Korpus:10 ↔ Tlok:10
- [Mate]: Korpus:10 ↔ Nakretka:10
- [Mate] (5 mm): Korpus:10 ↔ Nakretka:10
- Walcowe:10 [CylindricalJoint]: Korpus:10 ↔ Tlok:10
- [Mate]: Korpus:10 ↔ M5_70_shaft:10
- [Flush] (-32.5 mm): Korpus:10 ↔ M5_70_shaft:10
- [Mate]: M5_nut_5mm:64 ↔ M5_70_shaft:10
- [Mate]: M5_70_shaft:10 ↔ M5_nut_5mm:65
- [Mate] (60 mm): M5_nut_5mm:64 ↔ M5_nut_5mm:65
- [Mate] (27.5 mm): Korpus:10 ↔ M5_nut_5mm:64
- [Mate]: tuleja_TUF106040:72 ↔ ramie_1_wahacza:8
- [Mate]: tuleja_TUF106040:71 ↔ ramie_1_wahacza:8
- [Mate]: tuleja_TUF106040:72 ↔ ramie_1_wahacza:8
- [Mate]: tuleja_TUF106040:67 ↔ tuleja_TUF106040:73
- [Mate]: wspornik_amortyzatora:19 ↔ wspornik_amortyzatora:20
- [Mate]: wspornik_amortyzatora:19 ↔ wspornik_amortyzatora:20
- [Mate] (5 mm): wspornik_amortyzatora:19 ↔ wspornik_amortyzatora:20
- [Mate]: M3_16_shaft:10 ↔ wspornik_amortyzatora:20
- [Flush] (-2.5 mm): M3_16_shaft:10 ↔ wspornik_amortyzatora:19
- [Mate]: M3_16_shaft:10 ↔ M3_nut_2,5mm:19
- [Mate]: M3_nut_2,5mm:19 ↔ wspornik_amortyzatora:19
- [Mate]: M3_16_shaft:10 ↔ M3_nut_2,5mm:20
- [Mate]: M3_nut_2,5mm:20 ↔ wspornik_amortyzatora:20
- [Mate]: Tlok:10 ↔ M3_16_shaft:10
- [Mate]: Tlok:10 ↔ wspornik_amortyzatora:20
- [Mate]: ramie_1_wahacza:7 ↔ wspornik_amortyzatora:19
- [Mate]: ramie_1_wahacza:7 ↔ wspornik_amortyzatora:19
- [Mate] (4.5 mm): ramie_1_wahacza:7 ↔ wspornik_amortyzatora:19
- [Mate]: tuleja_TUF106040:70 ↔ M6_40_shaft:7
- [Flush] (7 mm): ramie_1_wahacza:7 ↔ M6_40_shaft:7
- [Mate]: tuleja_TUF106040:73 ↔ M6_40_shaft:8
- [Flush] (7 mm): ramie_2_wahacza:8 ↔ M6_40_shaft:8
- [Mate]: M6_nut_5mm:89 ↔ M6_40_shaft:7
- [Mate]: ramie_1_wahacza:7 ↔ M6_nut_5mm:89
- [Mate]: M6_40_shaft:7 ↔ M6_nut_5mm:90
- [Mate]: ramie_1_wahacza:8 ↔ M6_nut_5mm:90
- [Mate]: M6_40_shaft:8 ↔ M6_nut_5mm:91
- [Mate]: ramie_2_wahacza:7 ↔ M6_nut_5mm:91
- [Mate]: M6_40_shaft:8 ↔ M6_nut_5mm:92
- [Mate]: ramie_2_wahacza:8 ↔ M6_nut_5mm:92
- [Mate]: M6_40_shaft:7 ↔ tuleja_M6_M10_7:10
- [Mate]: M6_40_shaft:8 ↔ tuleja_M6_M10_7:11
- [Mate]: M6_1,25_pad:25 ↔ M6_1,25_pad:26
- [Mate]: M6_1,25_pad:25 ↔ M6_1,25_pad:26
- [Mate]: M6_40_shaft:7 ↔ M6_1,25_pad:25
- [Mate]: M6_1,25_pad:27 ↔ M6_1,25_pad:28
- [Mate]: M6_1,25_pad:27 ↔ M6_1,25_pad:28
- [Mate]: M6_40_shaft:7 ↔ M6_1,25_pad:27
- [Mate]: tuleja_TUF106040:70 ↔ M6_1,25_pad:27
- [Mate]: M6_1,25_pad:29 ↔ M6_1,25_pad:30
- [Mate]: M6_1,25_pad:29 ↔ M6_1,25_pad:30
- [Mate]: M6_40_shaft:8 ↔ M6_1,25_pad:29
- [Mate]: M6_1,25_pad:31 ↔ M6_1,25_pad:32
- [Mate]: M6_1,25_pad:31 ↔ M6_1,25_pad:32
- [Mate]: M6_40_shaft:8 ↔ M6_1,25_pad:31
- [Mate]: tuleja_TUF106040:73 ↔ M6_1,25_pad:31
- [Mate]: M5_70_shaft:10 ↔ M6_70_shaft:19
- [Flush]: M5_70_shaft:10 ↔ M6_70_shaft:20
- [Mate]: M6_70_shaft:20 ↔ M6_nut_5mm:93
- [Mate]: M6_70_shaft:20 ↔ M6_nut_5mm:94
- [Mate] (60 mm): M6_nut_5mm:93 ↔ M6_nut_5mm:94
- [Flush]: M5_nut_5mm:64 ↔ M6_nut_5mm:94
- [Mate] (60 mm): M6_nut_5mm:95 ↔ M6_nut_5mm:96
- [Mate]: M6_nut_5mm:95 ↔ M6_nut_5mm:96
- [Mate]: M6_70_shaft:19 ↔ M6_nut_5mm:95
- [Flush]: M5_nut_5mm:64 ↔ M6_nut_5mm:96
- [Mate]: ramie_1_wahacza:7 ↔ M5_shaft:7
- [Flush] (7 mm): ramie_1_wahacza:7 ↔ M5_shaft:7
- [Mate]: ramie_1_wahacza:7 ↔ M5_shaft:8
- [Flush] (7 mm): ramie_1_wahacza:7 ↔ M5_shaft:8
- [Mate]: M5_shaft:8 ↔ M5_nut_5mm:66
- [Mate]: ramie_1_wahacza:7 ↔ M5_nut_5mm:66
- [Mate]: M5_shaft:7 ↔ M5_nut_5mm:67
- [Mate]: ramie_1_wahacza:7 ↔ M5_nut_5mm:67
- [Mate]: M5_shaft:7 ↔ M5_nut_5mm:68
- [Mate]: ramie_1_wahacza:8 ↔ M5_nut_5mm:68
- [Mate]: M5_shaft:8 ↔ M5_nut_5mm:69
- [Mate]: ramie_1_wahacza:8 ↔ M5_nut_5mm:69
- [Mate]: M5_shaft:7 ↔ tuleja_M5_M9_4,5:13
- [Mate]: ramie_1_wahacza:8 ↔ tuleja_M5_M9_4,5:13
- [Mate]: M5_shaft:7 ↔ tuleja_M5_M9_4,5:14
- [Mate]: ramie_1_wahacza:7 ↔ tuleja_M5_M9_4,5:14
- [Mate]: M5_shaft:8 ↔ tuleja_M5_M9_4,5:15
- [Mate]: ramie_1_wahacza:8 ↔ tuleja_M5_M9_4,5:15
- [Mate]: M5_shaft:8 ↔ tuleja_M5_M9_4,5:16
- [Mate]: ramie_1_wahacza:7 ↔ tuleja_M5_M9_4,5:16
- [Mate]: M6_40_shaft:8 ↔ lacznik_zewn:7
- [Mate]: tuleja_M6_M10_7:11 ↔ lacznik_zewn:7
- [Mate]: M6_40_shaft:7 ↔ lacznik_zewn:7
- [Mate]: M6_40_shaft:8 ↔ lacznik_zewn:8
- [Mate]: M6_40_shaft:7 ↔ lacznik_zewn:8
- [Mate]: tuleja_TUF106040:72 ↔ M6_40_shaft:7
- [Mate]: M6_1,25_pad:28 ↔ lacznik_zewn:8
- [Mate]: M6_1,25_pad:32 ↔ lacznik_zewn:8
- [Mate]: tuleja_M6_M10_7:10 ↔ lacznik_zewn:7
- [Mate]: M6_1,25_pad:25 ↔ lacznik_zewn:7
- [Mate]: tuleja_TUF106040:72 ↔ M6_1,25_pad:26
- [Mate]: M6_1,25_pad:29 ↔ lacznik_zewn:7
- [Mate]: tuleja_TUF106040:67 ↔ M6_1,25_pad:30
- [Mate]: tuleja_TUF106040:71 ↔ ramie_1_wahacza:8
- [Mate]: tuleja_TUF106040:69 ↔ M6_70_shaft:20
- [Mate]: ramie_1_wahacza:7 ↔ tuleja_TUF106040:69
- [Mate]: ramie_1_wahacza:7 ↔ tuleja_TUF106040:69
- [Mate]: tuleja_TUF106040:68 ↔ M6_70_shaft:19
- [Mate]: ramie_2_wahacza:7 ↔ tuleja_TUF106040:68
- [Mate]: ramie_2_wahacza:7 ↔ tuleja_TUF106040:68
- [Mate]: tuleja_TUF106040:74 ↔ M6_70_shaft:19
- [Mate]: ramie_2_wahacza:8 ↔ tuleja_TUF106040:74
- [Mate]: ramie_2_wahacza:8 ↔ tuleja_TUF106040:74
- [Mate]: ramie_1_wahacza:8 ↔ M5_shaft:8
- [Mate]: M6_70_shaft:19 ↔ M6_nut_5mm:97
- [Mate] (5 mm): M6_nut_5mm:96 ↔ M6_nut_5mm:97
- [Mate]: M6_70_shaft:19 ↔ M6_nut_5mm:98
- [Mate] (5 mm): M6_nut_5mm:95 ↔ M6_nut_5mm:98
- [Mate]: M6_70_shaft:20 ↔ M6_nut_5mm:99
- [Mate] (5 mm): M6_nut_5mm:93 ↔ M6_nut_5mm:99
- [Mate]: M6_70_shaft:20 ↔ M6_nut_5mm:100
- [Mate] (5 mm): M6_nut_5mm:94 ↔ M6_nut_5mm:100
- [Mate]: M6_70_shaft:20 ↔ tuleja_M6_M10_6:13
- [Mate]: tuleja_M6_M10_6:13 ↔ M6_nut_5mm:99
- [Mate]: M6_70_shaft:19 ↔ tuleja_M6_M10_6:14
- [Mate]: tuleja_TUF106040:74 ↔ tuleja_M6_M10_6:14
- [Mate]: M6_70_shaft:19 ↔ tuleja_M6_M10_6:15
- [Mate]: tuleja_TUF106040:68 ↔ tuleja_M6_M10_6:15
- [Mate]: M6_70_shaft:20 ↔ tuleja_M6_M10_6:16
- [Mate]: tuleja_TUF106040:71 ↔ tuleja_M6_M10_6:16
- [Mate]: M5_70_shaft:10 ↔ M5_nut_5mm:70
- [Mate] (5 mm): M5_nut_5mm:64 ↔ M5_nut_5mm:70
- [Mate]: M5_70_shaft:10 ↔ M5_nut_5mm:71
- [Mate] (5 mm): M5_nut_5mm:65 ↔ M5_nut_5mm:71
- [Mate]: M5_70_shaft:10 ↔ tuleja_M5_M9_17.5:8
- [Mate]: M5_nut_5mm:71 ↔ tuleja_M5_M9_17.5:8
- [Mate]: M5_70_shaft:10 ↔ tuleja_M5_M9_17.5:7
- [Mate]: Korpus:10 ↔ tuleja_M5_M9_17.5:7
- Zestawiające:1632 [Mate]: plyta_boczna:1 ↔ M6_70_shaft:16
- Zestawiające:1633 [Mate]: plyta_boczna:1 ↔ M6_nut_5mm:75
- Zestawiające:1636 [Mate]: plyta_boczna:2 ↔ M6_70_shaft:15
- Zestawiające:1637 [Mate]: plyta_boczna:2 ↔ tuleja_M5_M9_17.5:3
- Kątowe:40 [Angle] (90 deg): ramie_1_wahacza:4 ↔ lacznik_zewn:3
- Zestawiające:1638 [Mate]: plyta_boczna:2 ↔ M5_nut_5mm:65
- Zestawiające:1639 [Mate]: plyta_boczna:2 ↔ M6_70_shaft:20
- Zestawiające:1640 [Mate]: plyta_boczna:2 ↔ M6_70_shaft:19
- Zestawiające:1641 [Mate]: plyta_boczna:2 ↔ tuleja_M5_M9_17.5:7
- Kątowe:41 [Angle] (90 deg): ramie_1_wahacza:7 ↔ lacznik_zewn:8
- [Mate]: ramie_2_wahacza:9 ↔ tuleja_TUF106040:75
- [Mate]: ramie_2_wahacza:9 ↔ tuleja_TUF106040:75
- [Angle] (0 deg): ramie_2_wahacza:9 ↔ tuleja_TUF106040:75
- [Mate]: ramie_1_wahacza:9 ↔ tuleja_TUF106040:78
- [Mate]: ramie_1_wahacza:9 ↔ tuleja_TUF106040:78
- [Angle] (0 deg): ramie_1_wahacza:9 ↔ tuleja_TUF106040:78
- [Mate]: ramie_2_wahacza:10 ↔ tuleja_TUF106040:81
- [Mate]: ramie_2_wahacza:10 ↔ tuleja_TUF106040:81
- [Angle] (0 deg): ramie_2_wahacza:10 ↔ tuleja_TUF106040:81
- [Mate]: Korpus:11 ↔ Tlok:11
- [Angle] (0 deg): Korpus:11 ↔ Tlok:11
- [Mate]: Korpus:11 ↔ Nakretka:11
- [Mate] (5 mm): Korpus:11 ↔ Nakretka:11
- Walcowe:11 [CylindricalJoint]: Korpus:11 ↔ Tlok:11
- [Mate]: Korpus:11 ↔ M5_70_shaft:11
- [Flush] (-32.5 mm): Korpus:11 ↔ M5_70_shaft:11
- [Mate]: M5_nut_5mm:72 ↔ M5_70_shaft:11
- [Mate]: M5_70_shaft:11 ↔ M5_nut_5mm:73
- [Mate] (60 mm): M5_nut_5mm:72 ↔ M5_nut_5mm:73
- [Mate] (27.5 mm): Korpus:11 ↔ M5_nut_5mm:72
- [Mate]: tuleja_TUF106040:80 ↔ ramie_1_wahacza:10
- [Mate]: tuleja_TUF106040:79 ↔ ramie_1_wahacza:10
- [Mate]: tuleja_TUF106040:80 ↔ ramie_1_wahacza:10